# Autodesk Inventor assembly: ExoskeletonV0p2
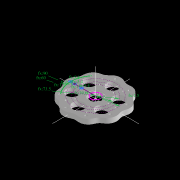
[picture p0: Inventor's stored thumbnail of the model, 180x180]
Saved by Autodesk Inventor 2022.2 (Build 262287010, 287A)
## iProperties
Created: 2022-05-24
Part Number: ExoskeletonV0p2
Document SubType Name: Assembly
Designer: Árni Þór Þorgeirsson
Author: Árni Þór Þorgeirsson
## Documents named in this file (4)
- G:\My Drive\Masters Thesis - exo\CAD_Files\ExoskeletonV0p2\ExoskeletonV0p2.iam
- G:\My Drive\Masters Thesis - exo\CAD_Files\ExoskeletonV0p2\Rotor_TSB\Top_Rotor_TSB.ipt
- G:\My Drive\Masters Thesis - exo\CAD_Files\ExoskeletonV0p2\Rotor_TSB\Bottom_Rotor_TSB.ipt
- G:\My Drive\Masters Thesis - exo\CAD_Files\ExoskeletonV0p2\Rotor_TSB\Rollers_Rotor_TSB.ipt
## Components (3 placed, 3 different names)
1. Top_Rotor_TSB:1 — Cylindrical:1, Insert:1, Flush:1, Flush:2, Flush:3
2. Bottom_Rotor_TSB:1 — Cylindrical:1, Insert:1
3. Rollers_Rotor_TSB:1 — Flush:1, Flush:2, Flush:3
## Relationships (5: Flush 3, CylindricalJoint 1, Insert 1)
- Cylindrical:1: Top_Rotor_TSB:1 ↔ Bottom_Rotor_TSB:1
- Insert:1: Top_Rotor_TSB:1 ↔ Bottom_Rotor_TSB:1
- Flush:1: Top_Rotor_TSB:1 ↔ Rollers_Rotor_TSB:1
- Flush:2: Top_Rotor_TSB:1 ↔ Rollers_Rotor_TSB:1
- Flush:3: Top_Rotor_TSB:1 ↔ Rollers_Rotor_TSB:1
